# Autodesk Inventor assembly: RR-PCSS-2021-2M2.1
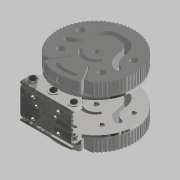
[picture p0: Inventor's stored thumbnail of the model, 180x180]
Saved by Autodesk Inventor 2021 (Build 250183000, 183)
## iProperties
Created: 2021-10-12
Part Number: RR-PCSS-2021-2M2.1
Document SubType Name: Assembly
Designer: marci
Author: marci
## Documents named in this file (7)
- C:\Users\marci\Desktop\Projekt ramienia\2M2\RR-PCSS-2021-2M2.1.iam
- C:\Users\marci\Desktop\Projekt ramienia\2M2\RR-PCSS-2021-W2M2MA1.ipt
- C:\Users\marci\Desktop\Projekt ramienia\2M2\RR-PCSS-2021-W2M2MA2.ipt
- C:\Users\marci\Desktop\Projekt ramienia\Nowy folder\pl-PL\ISO 4161\ISO 4161 - M5(1).ipt
- C:\Users\marci\Desktop\Projekt ramienia\Nowy folder\pl-PL\ISO 7380-1\ISO 7380-1 - M5 x 12.ipt
- C:\Users\marci\Desktop\Projekt ramienia\Nowy folder\pl-PL\ISO 7093 C\ISO 7093 C - ST 5 - 100 HV.ipt
- C:\Users\marci\Desktop\Projekt ramienia\2M2\RR-PCSS-2021-2M2.ipt
## Components (23 placed, 6 different names)
1. RR-PCSS-2021-W2M2MA1:1 — Zestawiające:1, Równoległe:1, Równoległe:4, Zestawiające:3, Równoległe:3, Równoległe:2, Zestawiające:4, Zestawiające:6, Zestawiające:8, Zestawiające:10, Zestawiające:11, Zestawiające:12, Zestawiające:13, Zestawiające:14, Zestawiające:15, Zestawiające:23, Zestawiające:25, Zestawiające:27
2. RR-PCSS-2021-W2M2MA2:1 — Zestawiające:1, Równoległe:1, Równoległe:4, Zestawiające:5, Zestawiające:7, Zestawiające:9, Wstawiające:8, Zestawiające:29, Symetria:1
3. RR-PCSS-2021-W2M2MA2:2 — Równoległe:2, Zestawiające:3, Równoległe:3, Zestawiające:16, Zestawiające:17, Zestawiające:18, Zestawiające:19, Zestawiające:20, Zestawiające:21, Zestawiające:22, Zestawiające:24, Zestawiające:26, Wstawiające:7, Zestawiające:28, Symetria:1
4. ISO 7380-1 M5 x 12:1 — Wstawiające:1
5. ISO 4161 M5:1 — Zestawiające:10, Zestawiające:11
6. ISO 7093 C ST 5 - 100 HV - C:1 — Zestawiające:4, Zestawiające:5, Wstawiające:1
7. ISO 7093 C ST 5 - 100 HV - C:2 — Zestawiające:6, Zestawiające:7, Wstawiające:2
8. ISO 7093 C ST 5 - 100 HV - C:3 — Zestawiające:8, Zestawiające:9, Wstawiające:3
9. ISO 7380-1 M5 x 12:2 — Wstawiające:2
10. ISO 7380-1 M5 x 12:3 — Wstawiające:3
11. ISO 4161 M5:2 — Zestawiające:12, Zestawiające:13
12. ISO 4161 M5:3 — Zestawiające:14, Zestawiające:15
13. ISO 7093 C ST 5 - 100 HV - C:4 — Zestawiające:16, Zestawiające:17, Wstawiające:4
14. ISO 7380-1 M5 x 12:4 — Wstawiające:4
15. ISO 4161 M5:4 — Zestawiające:22, Zestawiające:23
16. ISO 7093 C ST 5 - 100 HV - C:5 — Zestawiające:18, Zestawiające:19, Wstawiające:5
17. ISO 7093 C ST 5 - 100 HV - C:6 — Zestawiające:20, Zestawiające:21, Wstawiające:6
18. ISO 7380-1 M5 x 12:5 — Wstawiające:5
19. ISO 7380-1 M5 x 12:6 — Wstawiające:6
20. ISO 4161 M5:5 — Zestawiające:24, Zestawiające:25
21. ISO 4161 M5:6 — Zestawiające:26, Zestawiające:27
22. RR-PCSS-2021-2M2:1 — Wstawiające:7, Zestawiające:28
23. RR-PCSS-2021-2M2:2 — Wstawiające:8, Zestawiające:29
## Relationships (41: Mate 28, Insert 8, Flush 4, Symmetry 1)
- Zestawiające:1 [Mate]: RR-PCSS-2021-W2M2MA1:1 ↔ RR-PCSS-2021-W2M2MA2:1
- Równoległe:1 [Flush]: RR-PCSS-2021-W2M2MA1:1 ↔ RR-PCSS-2021-W2M2MA2:1
- Równoległe:4 [Flush]: RR-PCSS-2021-W2M2MA1:1 ↔ RR-PCSS-2021-W2M2MA2:1
- Równoległe:2 [Flush]: RR-PCSS-2021-W2M2MA1:1 ↔ RR-PCSS-2021-W2M2MA2:2
- Zestawiające:3 [Mate]: RR-PCSS-2021-W2M2MA1:1 ↔ RR-PCSS-2021-W2M2MA2:2
- Równoległe:3 [Flush]: RR-PCSS-2021-W2M2MA1:1 ↔ RR-PCSS-2021-W2M2MA2:2
- Zestawiające:4 [Mate]: RR-PCSS-2021-W2M2MA1:1 ↔ ISO 7093 C ST 5 - 100 HV - C:1
- Zestawiające:5 [Mate]: RR-PCSS-2021-W2M2MA2:1 ↔ ISO 7093 C ST 5 - 100 HV - C:1
- Zestawiające:6 [Mate]: RR-PCSS-2021-W2M2MA1:1 ↔ ISO 7093 C ST 5 - 100 HV - C:2
- Zestawiające:7 [Mate]: RR-PCSS-2021-W2M2MA2:1 ↔ ISO 7093 C ST 5 - 100 HV - C:2
- Zestawiające:8 [Mate]: RR-PCSS-2021-W2M2MA1:1 ↔ ISO 7093 C ST 5 - 100 HV - C:3
- Zestawiające:9 [Mate]: RR-PCSS-2021-W2M2MA2:1 ↔ ISO 7093 C ST 5 - 100 HV - C:3
- Wstawiające:1 [Insert]: ISO 7380-1 M5 x 12:1 ↔ ISO 7093 C ST 5 - 100 HV - C:1
- Wstawiające:2 [Insert]: ISO 7093 C ST 5 - 100 HV - C:2 ↔ ISO 7380-1 M5 x 12:2
- Wstawiające:3 [Insert]: ISO 7093 C ST 5 - 100 HV - C:3 ↔ ISO 7380-1 M5 x 12:3
- Zestawiające:10 [Mate]: RR-PCSS-2021-W2M2MA1:1 ↔ ISO 4161 M5:1
- Zestawiające:11 [Mate]: RR-PCSS-2021-W2M2MA1:1 ↔ ISO 4161 M5:1
- Zestawiające:12 [Mate]: RR-PCSS-2021-W2M2MA1:1 ↔ ISO 4161 M5:2
- Zestawiające:13 [Mate]: RR-PCSS-2021-W2M2MA1:1 ↔ ISO 4161 M5:2
- Zestawiające:14 [Mate]: RR-PCSS-2021-W2M2MA1:1 ↔ ISO 4161 M5:3
- Zestawiające:15 [Mate]: RR-PCSS-2021-W2M2MA1:1 ↔ ISO 4161 M5:3
- Zestawiające:16 [Mate]: RR-PCSS-2021-W2M2MA2:2 ↔ ISO 7093 C ST 5 - 100 HV - C:4
- Zestawiające:17 [Mate]: RR-PCSS-2021-W2M2MA2:2 ↔ ISO 7093 C ST 5 - 100 HV - C:4
- Zestawiające:18 [Mate]: RR-PCSS-2021-W2M2MA2:2 ↔ ISO 7093 C ST 5 - 100 HV - C:5
- Zestawiające:19 [Mate]: RR-PCSS-2021-W2M2MA2:2 ↔ ISO 7093 C ST 5 - 100 HV - C:5
- Zestawiające:20 [Mate]: RR-PCSS-2021-W2M2MA2:2 ↔ ISO 7093 C ST 5 - 100 HV - C:6
- Zestawiające:21 [Mate]: RR-PCSS-2021-W2M2MA2:2 ↔ ISO 7093 C ST 5 - 100 HV - C:6
- Wstawiające:4 [Insert]: ISO 7093 C ST 5 - 100 HV - C:4 ↔ ISO 7380-1 M5 x 12:4
- Wstawiające:5 [Insert]: ISO 7093 C ST 5 - 100 HV - C:5 ↔ ISO 7380-1 M5 x 12:5
- Wstawiające:6 [Insert]: ISO 7093 C ST 5 - 100 HV - C:6 ↔ ISO 7380-1 M5 x 12:6
- Zestawiające:22 [Mate]: RR-PCSS-2021-W2M2MA2:2 ↔ ISO 4161 M5:4
- Zestawiające:23 [Mate]: RR-PCSS-2021-W2M2MA1:1 ↔ ISO 4161 M5:4
- Zestawiające:24 [Mate]: RR-PCSS-2021-W2M2MA2:2 ↔ ISO 4161 M5:5
- Zestawiające:25 [Mate]: RR-PCSS-2021-W2M2MA1:1 ↔ ISO 4161 M5:5
- Zestawiające:26 [Mate]: RR-PCSS-2021-W2M2MA2:2 ↔ ISO 4161 M5:6
- Zestawiające:27 [Mate]: RR-PCSS-2021-W2M2MA1:1 ↔ ISO 4161 M5:6
- Wstawiające:7 [Insert]: RR-PCSS-2021-W2M2MA2:2 ↔ RR-PCSS-2021-2M2:1
- Wstawiające:8 [Insert]: RR-PCSS-2021-W2M2MA2:1 ↔ RR-PCSS-2021-2M2:2
- Zestawiające:28 [Mate]: RR-PCSS-2021-W2M2MA2:2 ↔ RR-PCSS-2021-2M2:1
- Zestawiające:29 [Mate]: RR-PCSS-2021-W2M2MA2:1 ↔ RR-PCSS-2021-2M2:2
- Symetria:1 [Symmetry]: RR-PCSS-2021-W2M2MA2:1 ↔ RR-PCSS-2021-W2M2MA2:2
